# Autodesk Inventor assembly: auth panel assembly
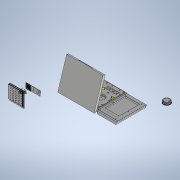
[picture p0: Inventor's stored thumbnail of the model, 180x180]
Saved by Autodesk Inventor 2022 (Build 260153000, 153)
## iProperties
Created: 2022-06-08
Part Number: auth panel assembly
Document SubType Name: Assembly
Designer: alecw
Author: alecw
## Documents named in this file (8)
- C:\aw_gd\Coding and Projects\smart home\smart-deadbolt\3D Modelling\auth panel assembly.iam
- C:\aw_gd\Coding and Projects\smart home\smart-deadbolt\3D Modelling\auth panel face plate seal.ipt
- C:\aw_gd\Coding and Projects\smart home\smart-deadbolt\3D Modelling\auth panel cover.ipt
- C:\aw_gd\Coding and Projects\smart home\smart-deadbolt\3D Modelling\auth panel face plate.ipt
- C:\aw_gd\Coding and Projects\smart home\smart-deadbolt\3D Modelling\keypad and cover.iam
- C:\aw_gd\Coding and Projects\smart home\smart-deadbolt\3D Modelling\1x3 button cover.ipt
- C:\aw_gd\Coding and Projects\smart home\smart-deadbolt\3D Modelling\authentication panel.ipt
- C:\aw_gd\Coding and Projects\smart home\smart-deadbolt\3D Modelling\fingerprint sensor.ipt
## Components (7 placed, 7 different names)
1. auth panel face plate seal:1 — Mate:1, Flush:1, Flush:2, Mate:2
2. auth panel cover:1 — Flush:5, Cylindrical:1
3. auth panel face plate:1 — Mate:2, Flush:3, Flush:4
4. keypad and cover:1 [sub-assembly]
5. 1x3 button cover:1
6. authentication panel:1 — Mate:1, Flush:1, Flush:2, Flush:3, Flush:4, Flush:5, Cylindrical:1
7. fingerprint sensor:1
## Relationships (8: Flush 5, Mate 2, CylindricalJoint 1)
- Mate:1: auth panel face plate seal:1 ↔ authentication panel:1
- Flush:1: auth panel face plate seal:1 ↔ authentication panel:1
- Flush:2: auth panel face plate seal:1 ↔ authentication panel:1
- Mate:2: auth panel face plate seal:1 ↔ auth panel face plate:1
- Flush:3: auth panel face plate:1 ↔ authentication panel:1
- Flush:4: auth panel face plate:1 ↔ authentication panel:1
- Flush:5: auth panel cover:1 ↔ authentication panel:1
- Cylindrical:1: auth panel cover:1 ↔ authentication panel:1
